# Autodesk Inventor assembly: dec_bot_design
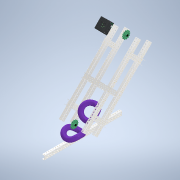
[picture p0: Inventor's stored thumbnail of the model, 180x180]
Saved by Autodesk Inventor 2022 (Build 260153000, 153)
## iProperties
Created: 2021-11-22
Part Number: dec_bot_design
Document SubType Name: Assembly
Designer: Alex
Author: Alex
## Documents named in this file (7)
- C:\Users\Alex\Documents\robotics\cad\DecBot\333B\dec_bot_design.iam
- C:\Users\Alex\Documents\robotics\cad\Library 1.2\Structure\C-Channels\Aluminum 1x2x1\1x2x1x35 Aluminum.ipt
- C:\Users\Alex\Documents\robotics\cad\Library 1.2\Electronics\V5 Motor.ipt
- C:\Users\Alex\Documents\robotics\cad\Tipping Poing Field CAD\Ring.ipt
- C:\Users\Alex\Documents\robotics\cad\Library 1.2\Structure\C-Channels\Aluminum 1x2x1\1x2x1x15 Aluminum.ipt
- C:\Users\Alex\Documents\robotics\cad\Library 1.2\Motion\Sprockets\HS 12T Sprocket, Square.ipt
- C:\Users\Alex\Documents\robotics\cad\Library 1.2\Structure\C-Channels\Aluminum 1x2x1\1x2x1x8 Aluminum.ipt
## Components (15 placed, 6 different names)
1. V5 Motor:1 — Insert:9, Insert:10
2. Ring:1
3. 1x2x1x15 Aluminum:1 — Insert:7, Insert:8, Insert:13, Insert:14
4. 1x2x1x35 Aluminum:3 — Insert:13, Insert:14, Insert:15, Insert:16, Insert:19, Insert:20
5. Ring:2
6. HS 12T Sprocket, Square:1 — Insert:12
7. HS 12T Sprocket, Square:2 — Insert:11
8. 1x2x1x35 Aluminum:4
9. 1x2x1x35 Aluminum:5 — Insert:7, Insert:8, Insert:9, Insert:10, Insert:11, Insert:12, Insert:23, Insert:24, Insert:25, Insert:26
10. 1x2x1x35 Aluminum:6 — Insert:17, Insert:18, Insert:21, Insert:22
11. 1x2x1x8 Aluminum:1 — Insert:15, Insert:16, Insert:17, Insert:18
12. 1x2x1x8 Aluminum:2 — Insert:19, Insert:20, Insert:21, Insert:22
13. 1x2x1x8 Aluminum:3 — Insert:23, Insert:24, Insert:27, Insert:28
14. 1x2x1x8 Aluminum:4 — Insert:25, Insert:26, Insert:29, Insert:30
15. 1x2x1x35 Aluminum:7 — Insert:27, Insert:28, Insert:29, Insert:30
## Relationships (24: Insert 24)
- Insert:7: 1x2x1x15 Aluminum:1 ↔ 1x2x1x35 Aluminum:5
- Insert:8: 1x2x1x15 Aluminum:1 ↔ 1x2x1x35 Aluminum:5
- Insert:9: V5 Motor:1 ↔ 1x2x1x35 Aluminum:5
- Insert:10: V5 Motor:1 ↔ 1x2x1x35 Aluminum:5
- Insert:11 (63.5 mm): HS 12T Sprocket, Square:2 ↔ 1x2x1x35 Aluminum:5
- Insert:12 (63.5 mm): HS 12T Sprocket, Square:1 ↔ 1x2x1x35 Aluminum:5
- Insert:13: 1x2x1x15 Aluminum:1 ↔ 1x2x1x35 Aluminum:3
- Insert:14: 1x2x1x15 Aluminum:1 ↔ 1x2x1x35 Aluminum:3
- Insert:15: 1x2x1x35 Aluminum:3 ↔ 1x2x1x8 Aluminum:1
- Insert:16: 1x2x1x35 Aluminum:3 ↔ 1x2x1x8 Aluminum:1
- Insert:17: 1x2x1x35 Aluminum:6 ↔ 1x2x1x8 Aluminum:1
- Insert:18: 1x2x1x35 Aluminum:6 ↔ 1x2x1x8 Aluminum:1
- Insert:19: 1x2x1x35 Aluminum:3 ↔ 1x2x1x8 Aluminum:2
- Insert:20: 1x2x1x35 Aluminum:3 ↔ 1x2x1x8 Aluminum:2
- Insert:21: 1x2x1x35 Aluminum:6 ↔ 1x2x1x8 Aluminum:2
- Insert:22: 1x2x1x35 Aluminum:6 ↔ 1x2x1x8 Aluminum:2
- Insert:23: 1x2x1x35 Aluminum:5 ↔ 1x2x1x8 Aluminum:3
- Insert:24: 1x2x1x35 Aluminum:5 ↔ 1x2x1x8 Aluminum:3
- Insert:25: 1x2x1x35 Aluminum:5 ↔ 1x2x1x8 Aluminum:4
- Insert:26: 1x2x1x35 Aluminum:5 ↔ 1x2x1x8 Aluminum:4
- Insert:27: 1x2x1x8 Aluminum:3 ↔ 1x2x1x35 Aluminum:7
- Insert:28: 1x2x1x8 Aluminum:3 ↔ 1x2x1x35 Aluminum:7
- Insert:29: 1x2x1x8 Aluminum:4 ↔ 1x2x1x35 Aluminum:7
- Insert:30: 1x2x1x8 Aluminum:4 ↔ 1x2x1x35 Aluminum:7
